# Autodesk Inventor assembly: Sessao_02_04_999_001
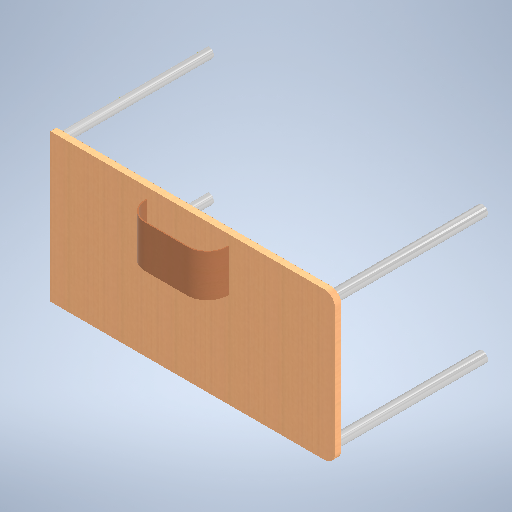
[picture p0: Inventor's stored thumbnail of the model, 512x512]
Saved by Autodesk Inventor 2026 (Build 300175000, 175)
## iProperties
Created: 2025-04-02
Part Number: Sessao_02_04_999_001
Document SubType Name: Assembly
Designer: Carlos Dias
Author: Carlos Dias
## Documents named in this file (4)
- C:\Users\Carlos Dias\Documents\Formação-TEARCI\UFCDs\5134 - Robótica _ Fundamentos\Material De Apoio\Sessao_02_04\Sessao_02_04_999_001.iam
- C:\Users\Carlos Dias\Documents\Formação-TEARCI\UFCDs\5134 - Robótica _ Fundamentos\Material De Apoio\Sessao_02_04\Sessao_02_04_001_001.ipt
- C:\Users\Carlos Dias\Documents\Formação-TEARCI\UFCDs\5134 - Robótica _ Fundamentos\Material De Apoio\Sessao_02_04\Sessao_02_04_002_001.ipt
- C:\Users\Carlos Dias\Documents\Formação-TEARCI\UFCDs\5134 - Robótica _ Fundamentos\Material De Apoio\Sessao_28_03\Sessao_28_03_003_001.ipt
## Components (6 placed, 3 different names)
1. Sessao_02_04_002_001:1 — Mate:1, Mate:2, Flush:1, Mate:4, Flush:11, Mate:5, Flush:12, Mate:6
2. Sessao_02_04_001_001:1 — Flush:4, Flush:5, Flush:6, Flush:7, Symmetry:1, Flush:8, Symmetry:2, Mate:4, Flush:11
3. Sessao_02_04_001_001:2 — Flush:4, Flush:7, Symmetry:1, Flush:10, Mate:6
4. Sessao_02_04_001_001:3 — Flush:5, Flush:8, Symmetry:2, Flush:9
5. Sessao_02_04_001_001:4 — Flush:6, Flush:9, Flush:10
6. Sessao_28_03_003_001:1 — Mate:5, Flush:12, Flush:13
## Relationships (18: Flush 11, Mate 5, Symmetry 2)
- Mate:1: Sessao_02_04_002_001:1
- Mate:2: Sessao_02_04_002_001:1
- Flush:1: Sessao_02_04_002_001:1
- Flush:4: Sessao_02_04_001_001:1 ↔ Sessao_02_04_001_001:2
- Flush:5: Sessao_02_04_001_001:1 ↔ Sessao_02_04_001_001:3
- Flush:6: Sessao_02_04_001_001:1 ↔ Sessao_02_04_001_001:4
- Flush:7: Sessao_02_04_001_001:1 ↔ Sessao_02_04_001_001:2
- Symmetry:1: Sessao_02_04_001_001:1 ↔ Sessao_02_04_001_001:2
- Flush:8: Sessao_02_04_001_001:1 ↔ Sessao_02_04_001_001:3
- Symmetry:2: Sessao_02_04_001_001:1 ↔ Sessao_02_04_001_001:3
- Flush:9: Sessao_02_04_001_001:3 ↔ Sessao_02_04_001_001:4
- Flush:10: Sessao_02_04_001_001:2 ↔ Sessao_02_04_001_001:4
- Mate:4 (-50 mm): Sessao_02_04_002_001:1 ↔ Sessao_02_04_001_001:1
- Flush:11 (50 mm): Sessao_02_04_002_001:1 ↔ Sessao_02_04_001_001:1
- Mate:5: Sessao_02_04_002_001:1 ↔ Sessao_28_03_003_001:1
- Flush:12 (50 mm): Sessao_02_04_002_001:1 ↔ Sessao_28_03_003_001:1
- Flush:13: Sessao_28_03_003_001:1
- Mate:6: Sessao_02_04_002_001:1 ↔ Sessao_02_04_001_001:2
